# Autodesk Inventor assembly: Square Coil
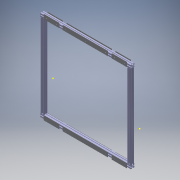
[picture p0: Inventor's stored thumbnail of the model, 180x180]
Saved by Autodesk Inventor 2019 (Build 230136000, 136)
## iProperties
Created: 2018-10-31
Part Number: Square Coil
Document SubType Name: Assembly
Designer: nomol
Author: nomol
## Documents named in this file (5)
- C:\Users\nomol\Downloads\Inventor\Helmholtz Cage\Square Coil.iam
- C:\Users\nomol\Downloads\Inventor\Helmholtz Cage\8020_TSlot_92cm.ipt
- C:\Users\nomol\Downloads\Inventor\Helmholtz Cage\8020_TSlot_1m.ipt
- C:\Users\nomol\Downloads\Inventor\Helmholtz Cage\Panel_5x17cm.ipt
- C:\Users\nomol\Downloads\Inventor\Helmholtz Cage\Panel_5x50cm.ipt
## Components (16 placed, 4 different names)
1. 8020_TSlot_1m:1 — Mate:1, Mate:2, Flush:1, Flush:3, Flush:6, Flush:7, Mate:4, Mate:5, Mate:6, Mate:7, Flush:9, Flush:10, Flush:11, Flush:12, Flush:13, Flush:14, Flush:15, Flush:16, Mate:8, Mate:9, Flush:17, Flush:18
2. 8020_TSlot_1m:2 — Mate:3, Flush:2, Flush:8, Mate:12, Mate:13, Mate:14, Mate:15, Mate:16, Mate:17, Flush:19, Flush:20, Flush:21, Flush:22, Flush:27, Flush:28, Flush:29, Flush:30, Flush:31, Flush:32
3. 8020_TSlot_92cm:1 — Mate:2, Flush:3, Flush:7, Flush:8
4. 8020_TSlot_92cm:2 — Mate:1, Mate:3, Flush:1, Flush:2, Flush:6
5. Panel_5x17cm:1 — Mate:4, Flush:11, Flush:16
6. Panel_5x17cm:2 — Mate:5, Flush:12, Flush:15
7. Panel_5x17cm:3 — Mate:7, Flush:9, Flush:14, Mate:10
8. Panel_5x17cm:4 — Mate:6, Flush:10, Flush:13, Mate:11
9. Panel_5x50cm:1 — Mate:9, Mate:10, Flush:18
10. Panel_5x50cm:2 — Mate:8, Mate:11, Flush:17
11. Panel_5x17cm:5 — Mate:13, Flush:21, Mate:19, Flush:31
12. Panel_5x17cm:6 — Mate:12, Flush:22, Mate:18, Flush:32
13. Panel_5x17cm:7 — Mate:14, Flush:20, Flush:30
14. Panel_5x17cm:8 — Mate:15, Flush:19, Flush:29
15. Panel_5x50cm:3 — Mate:17, Mate:19, Flush:27
16. Panel_5x50cm:4 — Mate:16, Mate:18, Flush:28
## Relationships (45: Flush 26, Mate 19)
- Mate:1: 8020_TSlot_1m:1 ↔ 8020_TSlot_92cm:2
- Mate:2: 8020_TSlot_1m:1 ↔ 8020_TSlot_92cm:1
- Mate:3: 8020_TSlot_1m:2 ↔ 8020_TSlot_92cm:2
- Flush:1: 8020_TSlot_1m:1 ↔ 8020_TSlot_92cm:2
- Flush:2: 8020_TSlot_1m:2 ↔ 8020_TSlot_92cm:2
- Flush:3: 8020_TSlot_1m:1 ↔ 8020_TSlot_92cm:1
- Flush:6: 8020_TSlot_1m:1 ↔ 8020_TSlot_92cm:2
- Flush:7: 8020_TSlot_1m:1 ↔ 8020_TSlot_92cm:1
- Flush:8: 8020_TSlot_1m:2 ↔ 8020_TSlot_92cm:1
- Mate:4: 8020_TSlot_1m:1 ↔ Panel_5x17cm:1
- Mate:5: 8020_TSlot_1m:1 ↔ Panel_5x17cm:2
- Mate:6: 8020_TSlot_1m:1 ↔ Panel_5x17cm:4
- Mate:7: 8020_TSlot_1m:1 ↔ Panel_5x17cm:3
- Flush:9 (40 mm): 8020_TSlot_1m:1 ↔ Panel_5x17cm:3
- Flush:10 (40 mm): 8020_TSlot_1m:1 ↔ Panel_5x17cm:4
- Flush:11 (40 mm): 8020_TSlot_1m:1 ↔ Panel_5x17cm:1
- Flush:12 (40 mm): 8020_TSlot_1m:1 ↔ Panel_5x17cm:2
- Flush:13: 8020_TSlot_1m:1 ↔ Panel_5x17cm:4
- Flush:14: 8020_TSlot_1m:1 ↔ Panel_5x17cm:3
- Flush:15: 8020_TSlot_1m:1 ↔ Panel_5x17cm:2
- Flush:16: 8020_TSlot_1m:1 ↔ Panel_5x17cm:1
- Mate:8: 8020_TSlot_1m:1 ↔ Panel_5x50cm:2
- Mate:9: 8020_TSlot_1m:1 ↔ Panel_5x50cm:1
- Mate:10 (40 mm): Panel_5x17cm:3 ↔ Panel_5x50cm:1
- Mate:11 (40 mm): Panel_5x17cm:4 ↔ Panel_5x50cm:2
- Flush:17: 8020_TSlot_1m:1 ↔ Panel_5x50cm:2
- Flush:18: 8020_TSlot_1m:1 ↔ Panel_5x50cm:1
- Mate:12: 8020_TSlot_1m:2 ↔ Panel_5x17cm:6
- Mate:13: 8020_TSlot_1m:2 ↔ Panel_5x17cm:5
- Mate:14: 8020_TSlot_1m:2 ↔ Panel_5x17cm:7
- Mate:15: 8020_TSlot_1m:2 ↔ Panel_5x17cm:8
- Mate:16: 8020_TSlot_1m:2 ↔ Panel_5x50cm:4
- Mate:17: 8020_TSlot_1m:2 ↔ Panel_5x50cm:3
- Flush:19 (40 mm): 8020_TSlot_1m:2 ↔ Panel_5x17cm:8
- Flush:20 (40 mm): 8020_TSlot_1m:2 ↔ Panel_5x17cm:7
- Flush:21 (40 mm): 8020_TSlot_1m:2 ↔ Panel_5x17cm:5
- Flush:22 (40 mm): 8020_TSlot_1m:2 ↔ Panel_5x17cm:6
- Mate:18 (40 mm): Panel_5x17cm:6 ↔ Panel_5x50cm:4
- Mate:19 (40 mm): Panel_5x17cm:5 ↔ Panel_5x50cm:3
- Flush:27: 8020_TSlot_1m:2 ↔ Panel_5x50cm:3
- Flush:28: 8020_TSlot_1m:2 ↔ Panel_5x50cm:4
- Flush:29: 8020_TSlot_1m:2 ↔ Panel_5x17cm:8
- Flush:30: 8020_TSlot_1m:2 ↔ Panel_5x17cm:7
- Flush:31: 8020_TSlot_1m:2 ↔ Panel_5x17cm:5
- Flush:32: 8020_TSlot_1m:2 ↔ Panel_5x17cm:6
